# Autodesk Inventor assembly: Assembly1
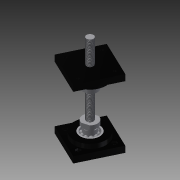
[picture p0: Inventor's stored thumbnail of the model, 180x180]
Saved by Autodesk Inventor 2015 (Build 190159000, 159)
## iProperties
Created: 2017-01-13
Part Number: Assembly1
Document SubType Name: Assembly
Designer: 1esh9
Author: 1esh9
## Documents named in this file (7)
- C:\Users\1esh9\Documents\Capstone-Project\doc\CAD\EndEffectorBase\Assembly1.iam
- C:\Users\1esh9\Documents\Capstone-Project\doc\CAD\EndEffectorBase\EEThreadedRod.ipt
- C:\Users\1esh9\Documents\Capstone-Project\doc\CAD\EndEffectorBase\BallBearingCone.ipt
- C:\Users\1esh9\Documents\Capstone-Project\doc\CAD\EndEffectorBase\BallBearingCup.ipt
- C:\Users\1esh9\Documents\Capstone-Project\doc\CAD\EndEffectorBase\BallBearing.ipt
- C:\Users\1esh9\Documents\Capstone-Project\doc\CAD\EndEffectorBase\BallBearingConeLockNut.ipt
- C:\Users\1esh9\Documents\Capstone-Project\doc\CAD\EndEffectorBase\BallBearingCupMount.ipt
## Components (11 placed, 6 different names)
1. EEThreadedRod:1 — Mate:1, Mate:2, Mate:3, Mate:4, Mate:5, Mate:6, Mate:7, Mate:10, Mate:11, Flush:1
2. BallBearingCone:1 — Mate:2, Mate:8, Mate:13
3. BallBearingCone:2 — Mate:3, Mate:9, Mate:12, Flush:1
4. BallBearingCup:1 — Mate:4, Tangent:1, Mate:8, Mate:16, Mate:17
5. BallBearingCup:2 — Mate:5, Tangent:2, Mate:9, Mate:14, Mate:15
6. BallBearing:1 — Mate:6, Tangent:1
7. BallBearing:2 — Mate:7, Tangent:2
8. BallBearingConeLockNut:1 — Mate:10, Mate:12
9. BallBearingConeLockNut:2 — Mate:11, Mate:13
10. BallBearingCupMount:1 — Mate:14, Mate:15, Flush:2
11. BallBearingCupMount:2 — Mate:16, Mate:17, Flush:2
## Relationships (21: Mate 17, Tangent 2, Flush 2)
- Mate:1: EEThreadedRod:1
- Mate:2: EEThreadedRod:1 ↔ BallBearingCone:1
- Mate:3: EEThreadedRod:1 ↔ BallBearingCone:2
- Mate:4: EEThreadedRod:1 ↔ BallBearingCup:1
- Mate:5: EEThreadedRod:1 ↔ BallBearingCup:2
- Mate:6: EEThreadedRod:1 ↔ BallBearing:1
- Mate:7: EEThreadedRod:1 ↔ BallBearing:2
- Tangent:1: BallBearingCup:1 ↔ BallBearing:1
- Mate:8 (-16.3 mm): BallBearingCone:1 ↔ BallBearingCup:1
- Tangent:2: BallBearingCup:2 ↔ BallBearing:2
- Mate:9 (-16.3 mm): BallBearingCone:2 ↔ BallBearingCup:2
- Mate:10: EEThreadedRod:1 ↔ BallBearingConeLockNut:1
- Mate:11: EEThreadedRod:1 ↔ BallBearingConeLockNut:2
- Mate:12: BallBearingCone:2 ↔ BallBearingConeLockNut:1
- Mate:13: BallBearingCone:1 ↔ BallBearingConeLockNut:2
- Flush:1: EEThreadedRod:1 ↔ BallBearingCone:2
- Mate:14: BallBearingCup:2 ↔ BallBearingCupMount:1
- Mate:15: BallBearingCup:2 ↔ BallBearingCupMount:1
- Mate:16: BallBearingCup:1 ↔ BallBearingCupMount:2
- Mate:17: BallBearingCup:1 ↔ BallBearingCupMount:2
- Flush:2: BallBearingCupMount:1 ↔ BallBearingCupMount:2
